# Autodesk Inventor assembly: OurWheelAssemblyBig_MIR
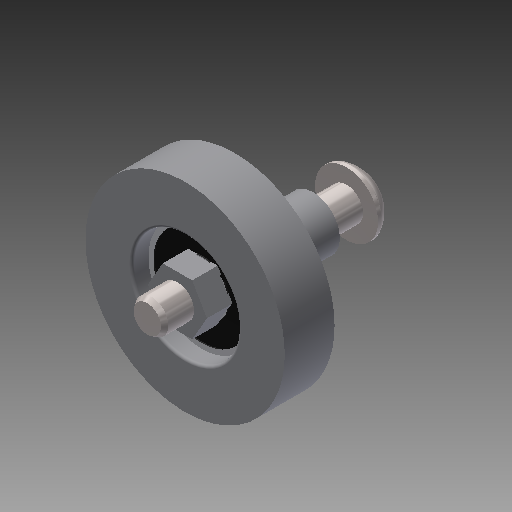
[picture p0: Inventor's stored thumbnail of the model, 512x512]
Saved by Autodesk Inventor 2017 (Build 210142000, 142)
## iProperties
Created: 2017-03-29
Part Number: OurWheelAssemblyBig_MIR
Document SubType Name: Assembly
Designer: umr
Author: umr
## Documents named in this file (6)
- D:\SeniorProject\Models2\WheelAssembly\OurWheelAssemblyBig_MIR.iam
- D:\SeniorProject\Models2\WheelAssembly\Precision Ball Bearing_MIR.ipt
- D:\SeniorProject\Models2\WheelAssembly\M5 Screw_30mm_MIR.ipt
- D:\SeniorProject\Models2\WheelAssembly\M5 Nut_MIR.ipt
- D:\SeniorProject\Models2\WheelAssembly\egzantrikNut_MIR.ipt
- D:\SeniorProject\Models2\WheelAssembly\Wheel_16-30_MIR.ipt
## Components (5 placed, 5 different names)
1. Precision Ball Bearing_MIR:1 — Mate:2, Mate:4, Mate:6, Mate:9, Mate:8
2. M5 Screw_30mm_MIR:1 — Mate:2, Mate:3, Mate:5, Mate:7
3. M5 Nut_MIR:1 — Mate:4, Mate:3
4. egzantrikNut_MIR:1 — Mate:5, Mate:6, Mate:7
5. Wheel_16-30_MIR:1 — Mate:9, Mate:8
## Relationships (8: Mate 8)
- Mate:2: Precision Ball Bearing_MIR:1 ↔ M5 Screw_30mm_MIR:1
- Mate:4: Precision Ball Bearing_MIR:1 ↔ M5 Nut_MIR:1
- Mate:3: M5 Screw_30mm_MIR:1 ↔ M5 Nut_MIR:1
- Mate:5: M5 Screw_30mm_MIR:1 ↔ egzantrikNut_MIR:1
- Mate:6: Precision Ball Bearing_MIR:1 ↔ egzantrikNut_MIR:1
- Mate:7 (5 mm): M5 Screw_30mm_MIR:1 ↔ egzantrikNut_MIR:1
- Mate:9: Precision Ball Bearing_MIR:1 ↔ Wheel_16-30_MIR:1
- Mate:8: Precision Ball Bearing_MIR:1 ↔ Wheel_16-30_MIR:1
